# Autodesk Inventor assembly: R2_D2
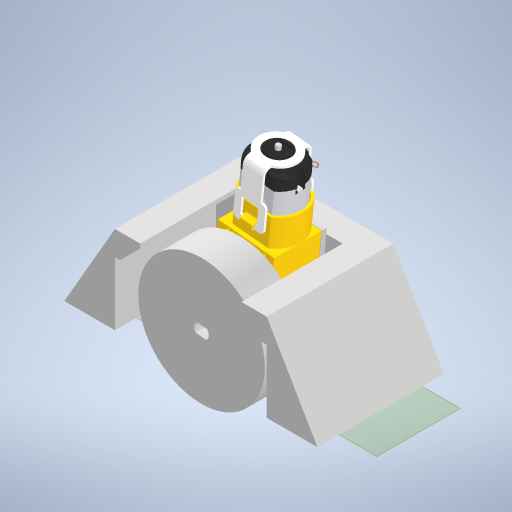
[picture p0: Inventor's stored thumbnail of the model, 512x512]
Saved by Autodesk Inventor 2024 (Build 280153000, 153)
## iProperties
Created: 2025-06-20
Part Number: R2_D2
Document SubType Name: Assembly
Designer: Aidan
Author: Aidan
## Documents named in this file (6)
- C:\Users\Aidan\OneDrive - University of New Haven\Documents\Fun Coding\R2-D2_V1\3D_Models\R2_D2.iam
- C:\Users\Aidan\OneDrive - University of New Haven\Documents\Fun Coding\R2-D2_V1\3D_Models\Wheel_well.ipt
- C:\Users\Aidan\OneDrive - University of New Haven\Documents\Fun Coding\R2-D2_V1\3D_Models\Skate-Bearing\Skate-Bearing.ipt
- C:\Users\Aidan\OneDrive - University of New Haven\Documents\Fun Coding\R2-D2_V1\3D_Models\motor_mount.ipt
- C:\Users\Aidan\OneDrive - University of New Haven\Documents\Fun Coding\R2-D2_V1\3D_Models\Mini Gear DC Motor 6 V Yellow\Mini Gear DC Motor 6 V Yellow.ipt
- C:\Users\Aidan\OneDrive - University of New Haven\Documents\Fun Coding\R2-D2_V1\3D_Models\Wheel.ipt
## Components (5 placed, 5 different names)
1. Wheel_well:1 — Insert:1
2. Skate-Bearing:1 — Insert:1, Rotational:1
3. motor_mount:1 — Rotational:1, Mate:1, Flush:3, Flush:4
4. Mini Gear DC Motor 6 V Yellow:1 — Mate:1, Flush:3, Flush:4, Mate:2
5. Wheel:1 — Mate:2
## Relationships (6: Mate 2, Flush 2, Insert 1, RevoluteJoint 1)
- Insert:1: Wheel_well:1 ↔ Skate-Bearing:1
- Rotational:1 [RevoluteJoint] (-7 mm): Skate-Bearing:1 ↔ motor_mount:1
- Mate:1: motor_mount:1 ↔ Mini Gear DC Motor 6 V Yellow:1
- Flush:3: motor_mount:1 ↔ Mini Gear DC Motor 6 V Yellow:1
- Flush:4: motor_mount:1 ↔ Mini Gear DC Motor 6 V Yellow:1
- Mate:2: Mini Gear DC Motor 6 V Yellow:1 ↔ Wheel:1
